# Autodesk Inventor assembly: main
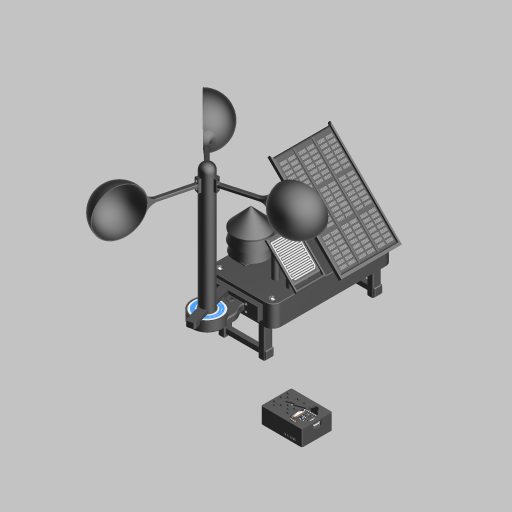
[picture p0: Inventor's stored thumbnail of the model, 512x512]
Saved by Autodesk Inventor 2024.4 (Build 284460000, 460)
## iProperties
Created: 2026-02-13
Part Number: main
Document SubType Name: Assembly
Designer: User
Author: User
## Documents named in this file (30)
- C:\Users\Duszy\Desktop\Projekty\Pogodynka\Model\main.iam
- C:\Users\Duszy\Desktop\Projekty\Pogodynka\Model\Stacja\spod.ipt
- C:\Users\Duszy\Desktop\Projekty\Pogodynka\Model\Stacja\gora.ipt
- C:\Users\Duszy\Desktop\Projekty\Pogodynka\Model\Stacja\anomierz_rama.ipt
- C:\Users\Duszy\Desktop\Projekty\Pogodynka\Model\Stacja\p  BEARING, SINGLE-ROW RADIAL, DOUBLE-SEALED, METRIC 6000-2RS SERIES  —  6004-2RS — 20mm ID × 42mm OD × 12mm W\p  BEARING, SINGLE-ROW RADIAL, DOUBLE-SEALED, METRIC 6000-2R.ipt
- C:\Users\Duszy\Desktop\Projekty\Pogodynka\Model\Stacja\andomierz_wal.ipt
- C:\Users\Duszy\Desktop\Projekty\Pogodynka\Model\Stacja\czasza.ipt
- C:\Users\Duszy\Desktop\Projekty\Pogodynka\Model\Stacja\solar_stand.ipt
- C:\Users\Duszy\Desktop\Projekty\Pogodynka\Model\Stacja\watrer_stand.ipt
- C:\Users\Duszy\Desktop\Projekty\Pogodynka\Model\Stacja\sensor_holder.ipt
- C:\Users\Duszy\Desktop\Projekty\Pogodynka\Model\Stacja\ul.ipt
- C:\Users\Duszy\Desktop\Projekty\Pogodynka\Model\Stacja\tarcza_wal.ipt
- C:\Users\Duszy\Desktop\Projekty\Pogodynka\Model\Stacja\clamp.ipt
- C:\Users\Duszy\Desktop\Projekty\Pogodynka\Model\Odbiornik\Odbiornik_bot.ipt
- C:\Users\Duszy\Desktop\Projekty\Pogodynka\Model\Odbiornik\Odbiornik_top.ipt
- C:\Users\Duszy\Desktop\Projekty\Pogodynka\Model\Stacja\kołek.ipt
- C:\Users\Duszy\Desktop\Projekty\Pogodynka\Model\Stacja\UL2.ipt
- C:\Users\Duszy\Desktop\Projekty\Pogodynka\Model\hoja v2\hoja v2\hoja v2.ipt
- C:\Users\Duszy\Desktop\Projekty\Pogodynka\Model\SolarPanel_30x65x3mm\SolarPanel_30x65x3mm\SolarPanel_30x65x3mm.ipt
- C:\Users\Duszy\Desktop\Projekty\Pogodynka\Model\ESP32 WROOM\ESP32 WROOM\ESP32 WROOM.ipt
- C:\Users\Duszy\Desktop\Projekty\Pogodynka\Model\ESP32 WROOM\97164A115_Aluminum Tapered Heat-Set Inserts for Plastic\97164A115_Aluminum Tapered Heat-Set Inserts for Plastic.ipt
- C:\Users\Duszy\Desktop\Projekty\Pogodynka\Model\ESP32 WROOM\92000A228_Passivated 18-8 Stainless Steel Pan Head Phillips Screws\92000A228_Passivated 18-8 Stainless Steel Pan Head Phillips Screws.ipt
- C:\Users\Duszy\Desktop\Projekty\Pogodynka\Model\Stacja\main\AIP\FEA\fc5dssn29.fres
- C:\Users\Duszy\Desktop\Projekty\Pogodynka\Model\Stacja\main\AIP\FEA\fc5hcz1s1.fres
- C:\Users\Duszy\Desktop\Projekty\Pogodynka\Model\main\AIP\FEA\fc5dssmzk.fins
- C:\Users\Duszy\Desktop\Projekty\Pogodynka\Model\main\AIP\FEA\fc5dssmzk.fsat
- C:\Users\Duszy\Desktop\Projekty\Pogodynka\Model\main\AIP\FEA\fc5dssmzk.ftes
- C:\Users\Duszy\Desktop\Projekty\Pogodynka\Model\main\AIP\FEA\fc5dssmzk.fwiz
- C:\Users\Duszy\Desktop\Projekty\Pogodynka\Model\main\AIP\FEA\fc5dssn28.fmsh
- C:\Users\Duszy\Desktop\Projekty\Pogodynka\Model\main\AIP\FEA\fdf1yomqo.fres
## Components (39 placed, 21 different names)
1. spod:1 — Obrotowe:11, Obrotowe:12, Obrotowe:13, Obrotowe:14, Obrotowe:15, Obrotowe:16, Obrotowe:22
2. gora:1 — Sztywne:2, Obrotowe:5, Obrotowe:15, Obrotowe:16, Obrotowe:17, Obrotowe:20, Obrotowe:23
3. anomierz_rama:1 — Obrotowe:9, Obrotowe:13, Obrotowe:14
4. p  BEARING, SINGLE-ROW RADIAL, DOUBLE-SEALED, METRIC 6000-2R:1 — Obrotowe:8, Obrotowe:9
5. andomierz_wal:1 — Obrotowe:4, Obrotowe:8, Obrotowe:10
6. solar_stand:1 — Sztywne:2, Sztywne:4
7. watrer_stand:1 — Obrotowe:5, Obrotowe:17, Sztywne:6
8. sensor_holder:1 — Obrotowe:20, Obrotowe:21
9. ul:1
10. tarcza_wal:1 — Obrotowe:10
11. clamp:1 — Obrotowe:11
12. clamp:2 — Obrotowe:12, Sztywne:3
13. Odbiornik_bot:1 — Obrotowe:19, Sztywne:5
14. Odbiornik_top:1 — Obrotowe:19
15. UL2:1 — Obrotowe:21
16. hoja v2:1 — Sztywne:6
17. ESP32 WROOM:1 — Sztywne:5
18. czasza:1 — Obrotowe:4
19. czasza:2
20. czasza:3
21. kołek:1 — Sztywne:3
22. kołek:2
23. SolarPanel_30x65x3mm:1 — Sztywne:4
24. SolarPanel_30x65x3mm:2
25. SolarPanel_30x65x3mm:3
26. SolarPanel_30x65x3mm:4
27. SolarPanel_30x65x3mm:5
28. SolarPanel_30x65x3mm:6
29. SolarPanel_30x65x3mm:7
30. SolarPanel_30x65x3mm:8
31. SolarPanel_30x65x3mm:9
32. 92000A228_Passivated 18-8 Stainless Steel Pan Head Phillips Screws:1 — Obrotowe:23
33. 97164A115_Aluminum Tapered Heat-Set Inserts for Plastic:1 — Obrotowe:22
34. 92000A228_Passivated 18-8 Stainless Steel Pan Head Phillips Screws:2
35. 97164A115_Aluminum Tapered Heat-Set Inserts for Plastic:2
36. 92000A228_Passivated 18-8 Stainless Steel Pan Head Phillips Screws:3
37. 97164A115_Aluminum Tapered Heat-Set Inserts for Plastic:3
38. 92000A228_Passivated 18-8 Stainless Steel Pan Head Phillips Screws:4
39. 97164A115_Aluminum Tapered Heat-Set Inserts for Plastic:4
## Component patterns: (3 elements, first: czasza:1), (2 elements, first: kołek:1), (9 elements, first: SolarPanel_30x65x3mm:1), (4 elements, first: 92000A228_Passivated 18-8 Stainless Steel Pan Head Phillips Screws:1 + 97164A115_Aluminum Tapered Heat-Set Inserts for Plastic:1)
## Relationships (22: RevoluteJoint 17, WeldJoint 5)
- Obrotowe:4 [RevoluteJoint] (3 mm): andomierz_wal:1 ↔ czasza:1
- Sztywne:2 [WeldJoint]: gora:1 ↔ solar_stand:1
- Obrotowe:5 [RevoluteJoint]: gora:1 ↔ watrer_stand:1
- Obrotowe:8 [RevoluteJoint]: p  BEARING, SINGLE-ROW RADIAL, DOUBLE-SEALED, METRIC 6000-2R:1 ↔ andomierz_wal:1
- Obrotowe:9 [RevoluteJoint] (-6 mm): anomierz_rama:1 ↔ p  BEARING, SINGLE-ROW RADIAL, DOUBLE-SEALED, METRIC 6000-2R:1
- Obrotowe:10 [RevoluteJoint]: andomierz_wal:1 ↔ tarcza_wal:1
- Obrotowe:11 [RevoluteJoint]: spod:1 ↔ clamp:1
- Obrotowe:12 [RevoluteJoint]: spod:1 ↔ clamp:2
- Obrotowe:13 [RevoluteJoint]: spod:1 ↔ anomierz_rama:1
- Obrotowe:14 [RevoluteJoint]: spod:1 ↔ anomierz_rama:1
- Obrotowe:15 [RevoluteJoint]: spod:1 ↔ gora:1
- Obrotowe:16 [RevoluteJoint]: spod:1 ↔ gora:1
- Obrotowe:17 [RevoluteJoint]: gora:1 ↔ watrer_stand:1
- Obrotowe:19 [RevoluteJoint]: Odbiornik_bot:1 ↔ Odbiornik_top:1
- Sztywne:3 [WeldJoint] (0.2 mm): clamp:2 ↔ kołek:1
- Obrotowe:20 [RevoluteJoint] (-1.1 mm): gora:1 ↔ sensor_holder:1
- Obrotowe:21 [RevoluteJoint] (-0.1 mm): sensor_holder:1 ↔ UL2:1
- Sztywne:4 [WeldJoint] (26 mm): solar_stand:1 ↔ SolarPanel_30x65x3mm:1
- Sztywne:5 [WeldJoint] (4 mm): Odbiornik_bot:1 ↔ ESP32 WROOM:1
- Sztywne:6 [WeldJoint] (-50 mm): watrer_stand:1 ↔ hoja v2:1
- Obrotowe:22 [RevoluteJoint] (-4.7 mm): spod:1 ↔ 97164A115_Aluminum Tapered Heat-Set Inserts for Plastic:1
- Obrotowe:23 [RevoluteJoint] (19 mm): gora:1 ↔ 92000A228_Passivated 18-8 Stainless Steel Pan Head Phillips Screws:1
## Named parameters: sa_0 = 981, sa_4 = 100, sa_5 = 981, sa_6 = 100, sa_7 = 10000, sa_8 = 10000, sa_9 = 10000, sa_1 = 1000, sa_2 = 1000, sa_3 = 1000
note: some values were not read from the file. Shown as the stored number, unit unknown: "sa_0", "sa_4", "sa_5", "sa_6", "sa_7", "sa_8", "sa_9", "sa_1", "sa_2", "sa_3".
